# Autodesk Inventor assembly: Flex_Giubo_Assembly
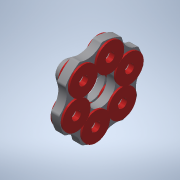
[picture p0: Inventor's stored thumbnail of the model, 180x180]
Saved by Autodesk Inventor 2021 (Build 250183000, 183)
## iProperties
Created: 2020-10-13
Part Number: Flex_Giubo_Assembly
Document SubType Name: Assembly
Designer: PhotonUser
Quantity: 1
Author: PhotonUser
## Documents named in this file (4)
- D:\PhotonUser\Downloads\Assembly Files-20201012T234257Z-001\Assembly Files\Flex_Giubo_Assembly.iam
- D:\PhotonUser\Downloads\Assembly Files-20201012T234257Z-001\Assembly Files\Poly_Bushing.ipt
- D:\PhotonUser\Downloads\Assembly Files-20201012T234257Z-001\Assembly Files\Flex_Giubo_V1.ipt
- D:\PhotonUser\Downloads\Assembly Files-20201012T234257Z-001\Assembly Files\Torque_Triangle.ipt
## Components (14 placed, 3 different names)
1. Poly_Bushing:1 — Insert:4
2. Poly_Bushing:2 — Insert:10
3. Poly_Bushing:3 — Insert:6, Insert:14
4. Poly_Bushing:4 — Insert:3
5. Poly_Bushing:5 — Insert:2
6. Poly_Bushing:6 — Insert:1
7. Poly_Bushing:7 — Insert:7
8. Poly_Bushing:8 — Insert:8
9. Poly_Bushing:9 — Insert:9
10. Poly_Bushing:10 — Insert:11
11. Poly_Bushing:11 — Insert:12
12. Poly_Bushing:12 — Insert:5
13. Flex_Giubo_V1:1 — Insert:1, Insert:2, Insert:3, Insert:4, Insert:5, Insert:6, Insert:7, Insert:8, Insert:9, Insert:10, Insert:11, Insert:12, Insert:13
14. Torque_Triangle:1 — Insert:13, Insert:14
## Relationships (14: Insert 14)
- Insert:1: Poly_Bushing:6 ↔ Flex_Giubo_V1:1
- Insert:2: Poly_Bushing:5 ↔ Flex_Giubo_V1:1
- Insert:3: Poly_Bushing:4 ↔ Flex_Giubo_V1:1
- Insert:4: Poly_Bushing:1 ↔ Flex_Giubo_V1:1
- Insert:5: Poly_Bushing:12 ↔ Flex_Giubo_V1:1
- Insert:6: Poly_Bushing:3 ↔ Flex_Giubo_V1:1
- Insert:7: Poly_Bushing:7 ↔ Flex_Giubo_V1:1
- Insert:8: Poly_Bushing:8 ↔ Flex_Giubo_V1:1
- Insert:9: Poly_Bushing:9 ↔ Flex_Giubo_V1:1
- Insert:10: Poly_Bushing:2 ↔ Flex_Giubo_V1:1
- Insert:11: Poly_Bushing:10 ↔ Flex_Giubo_V1:1
- Insert:12: Poly_Bushing:11 ↔ Flex_Giubo_V1:1
- Insert:13 (1.999 mm): Flex_Giubo_V1:1 ↔ Torque_Triangle:1
- Insert:14: Poly_Bushing:3 ↔ Torque_Triangle:1
